# Autodesk Inventor assembly: roller
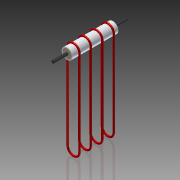
[picture p0: Inventor's stored thumbnail of the model, 180x180]
Saved by Autodesk Inventor 2011 SP1 (Build 150282100, 282)
## iProperties
Created: 2012-01-20
Part Number: roller
Document SubType Name: Assembly
Designer: Christopher
Author: Christopher
## Documents named in this file (6)
- C:\Users\Christopher\Documents\Christopher\FIRST\Inventor files\2012\tower bottom second design\roller.iam
- C:\Users\Christopher\Documents\Christopher\FIRST\Inventor files\2012\tower bottom second design\8 in pvc roller 1.379.ipt
- C:\Users\Christopher\Documents\Christopher\FIRST\Inventor files\2012\tower bottom second design\13 in axle.ipt
- C:\Users\Christopher\Documents\Christopher\FIRST\Inventor files\2012\tower bottom second design\axlebracetopvc.ipt
- C:\Users\Christopher\Documents\Christopher\FIRST\Inventor files\2012\tower bottom second design\14in polycord loop.ipt
- C:\Users\Christopher\Documents\Christopher\FIRST\Inventor files\2012\tower bottom second design\14 inch polycord 1.1.ipt
## Components (12 placed, 5 different names)
1. 8 in pvc roller 1.379:1 — Insert:1, Insert:2, Insert:4, Insert:5, Insert:6, Insert:7, Insert:8, Insert:9, Insert:10, Insert:11, Insert:12, Insert:13, Insert:15
2. 13 in axle:1 — Insert:3
3. axlebracetopvc:1 — Insert:1
4. axlebracetopvc:2 — Insert:2, Insert:3, Insert:14
5. 14in polycord loop:1 — Insert:4
6. 14in polycord loop:2 — Insert:5
7. 14in polycord loop:3 — Insert:6
8. 14in polycord loop:4 — Insert:7
9. 14 inch polycord 1.1:1 — Insert:11, Flush:1, Insert:12
10. 14 inch polycord 1.1:2 — Insert:10, Flush:1, Flush:2, Insert:13
11. 14 inch polycord 1.1:3 — Insert:9, Flush:2, Flush:3, Insert:14
12. 14 inch polycord 1.1:4 — Insert:8, Flush:3, Insert:15
## Relationships (18: Insert 15, Flush 3)
- Insert:1: 8 in pvc roller 1.379:1 ↔ axlebracetopvc:1
- Insert:2: 8 in pvc roller 1.379:1 ↔ axlebracetopvc:2
- Insert:3 (63.5 mm): 13 in axle:1 ↔ axlebracetopvc:2
- Insert:4 (25.4 mm): 8 in pvc roller 1.379:1 ↔ 14in polycord loop:1
- Insert:5 (76.2 mm): 8 in pvc roller 1.379:1 ↔ 14in polycord loop:2
- Insert:6 (127 mm): 8 in pvc roller 1.379:1 ↔ 14in polycord loop:3
- Insert:7 (177.8 mm): 8 in pvc roller 1.379:1 ↔ 14in polycord loop:4
- Insert:8 (25.4 mm): 8 in pvc roller 1.379:1 ↔ 14 inch polycord 1.1:4
- Insert:9 (76.2 mm): 8 in pvc roller 1.379:1 ↔ 14 inch polycord 1.1:3
- Insert:10 (127 mm): 8 in pvc roller 1.379:1 ↔ 14 inch polycord 1.1:2
- Insert:11 (177.8 mm): 8 in pvc roller 1.379:1 ↔ 14 inch polycord 1.1:1
- Flush:1: 14 inch polycord 1.1:1 ↔ 14 inch polycord 1.1:2
- Flush:2: 14 inch polycord 1.1:2 ↔ 14 inch polycord 1.1:3
- Flush:3: 14 inch polycord 1.1:3 ↔ 14 inch polycord 1.1:4
- Insert:12 (25.4 mm): 8 in pvc roller 1.379:1 ↔ 14 inch polycord 1.1:1
- Insert:13 (76.2 mm): 8 in pvc roller 1.379:1 ↔ 14 inch polycord 1.1:2
- Insert:14 (127 mm): axlebracetopvc:2 ↔ 14 inch polycord 1.1:3
- Insert:15 (177.8 mm): 8 in pvc roller 1.379:1 ↔ 14 inch polycord 1.1:4
